# Autodesk Inventor assembly: CoreXY_Unit_Asem
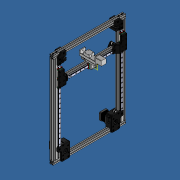
[picture p0: Inventor's stored thumbnail of the model, 180x180]
Saved by Autodesk Inventor 2020 (Build 240168000, 168)
## iProperties
Created: 2020-09-22
Part Number: CoreXY_Unit_Asem
Document SubType Name: Assembly
Designer: magnarecta
Author: magnarecta
## Documents named in this file (28)
- D:\Document\Github\CoreXY_Laser\Model\Asem\CoreXY_Unit_Asem.iam
- D:\Document\Github\CoreXY_Laser\Model\Parts\Linear_Guide\MGN12H_400mm\MGN12H_400mm.iam
- D:\Document\Github\CoreXY_Laser\Model\Parts\MISUMI\HFS5-2020-300_Autodesk_Inventor_2020_20200923\HFS5-2020-300.ipt
- D:\Document\Github\CoreXY_Laser\Model\Parts\MISUMI\HFS5-2020-420-Z5-XA10-XB30-XC390-XD410_Autodesk_Inventor_2020_20200923\HFS5-2020-420-Z5-XA10-XB30-XC390-XD410.ipt
- D:\Document\Github\CoreXY_Laser\Model\Parts\Stepper Motor\NEMA17\17HS4401\17HS4401S.ipt
- D:\Document\Github\CoreXY_Laser\Model\Parts\Idler\GT2\GT2 Pulley 20T 5mm bore without\GT2 idler pulley (5 mm bore) .ipt
- D:\Document\Github\CoreXY_Laser\Model\Parts\Pulley\GT2\GT2_20t\GT2_20teeth_5bore.ipt
- D:\Document\Github\CoreXY_Laser\Model\Parts\Print_Parts\Print_Parts_C.ipt
- D:\Document\Github\CoreXY_Laser\Model\Parts\Print_Parts\Print_Parts_D.ipt
- D:\Document\Github\CoreXY_Laser\Model\Parts\Print_Parts\Print_Parts_E.ipt
- D:\Document\Github\CoreXY_Laser\Model\Parts\Print_Parts\Print_Parts_F.ipt
- D:\Document\Github\CoreXY_Laser\Model\Parts\Print_Parts\Print_Parts_I.ipt
- D:\Document\Github\CoreXY_Laser\Model\Parts\Print_Parts\Print_Parts_J.ipt
- D:\Document\Github\CoreXY_Laser\Model\Parts\MISUMI\HFS5-2020-420-AV63.5-BV356.5-Z5-XA10-XB30-XC390-XD410_Autodesk_Inventor_2020_20201005\HFS5-2020-420-AV63_5-BV356_5-Z5-XA10-XB30-XC390-XD410.ipt
- D:\Document\Github\CoreXY_Laser\Model\Parts\Bolt\M5 x 20.ipt
- D:\Document\Github\CoreXY_Laser\Model\Parts\Bolt\M3 x 8.ipt
- D:\Document\Github\CoreXY_Laser\Model\Parts\Bolt\M4 x 8.ipt
- D:\Document\Github\CoreXY_Laser\Model\Parts\Bolt\M3 x 25.ipt
- D:\Document\Github\CoreXY_Laser\Model\Parts\Bolt\M3 x 30.ipt
- D:\Document\Github\CoreXY_Laser\Model\Parts\Bolt\M4 x 10.ipt
- D:\Document\Github\CoreXY_Laser\Model\Parts\Bolt\M3 x 35.ipt
- D:\Document\Github\CoreXY_Laser\Model\Parts\Bolt\M3 x 40.ipt
- D:\Document\Github\CoreXY_Laser\Model\Parts\MISUMI\HFS5-2040-510_Autodesk_Inventor_2020_20210519\HFS5-2040-510.ipt
- D:\Document\Github\CoreXY_Laser\Model\Parts\Print_Parts\Rev3_Parts\CoreXY_A.ipt
- D:\Document\Github\CoreXY_Laser\Model\Parts\Print_Parts\Rev3_Parts\CoreXY_B.ipt
- D:\Document\Github\CoreXY_Laser\Model\Parts\Linear_Guide\MGN12H_250mm\MGN12H_250mm.iam
- D:\Document\Github\CoreXY_Laser\Model\Parts\Linear_Guide\Linear_Unit\Linear_Unit.iam
- D:\Document\Github\CoreXY_Laser\Model\Parts\Print_Parts\Rev3_Parts\Linear_Unit_Mount.ipt
## Components (87 placed, 27 different names)
1. HFS5-2040-510:1 — 角度:5
2. MGN12H_400mm:2 [sub-assembly] — Mate:4, Flush:7, Insert:122, メイト:163, 挿入:178, メイト:170, メイト:171
3. HFS5-2040-510:2
4. MGN12H_400mm:3 [sub-assembly] — Mate:30, Flush:7, Insert:119, Insert:120, 挿入:179, メイト:172
5. HFS5-2020-420-Z5-XA10-XB30-XC390-XD410:1 — Insert:30, Insert:31, Insert:32, Insert:33, メイト:158, メイト:161
6. GT2 idler pulley (5 mm bore) :11 — Mate:70, フラッシュ:36
7. Print_Parts_J:1 — Flush:32, メイト:118, メイト:119, フラッシュ:49, Insert:82, Insert:83, Insert:84, Insert:88, Insert:89, Insert:90, Insert:134
8. Print_Parts_J:2 — Flush:32, メイト:116, メイト:117, フラッシュ:48, フラッシュ:49, Insert:85, Insert:86, Insert:87, Insert:91, Insert:92, Insert:93, Insert:135
9. Print_Parts_I:3 — Mate:70, Flush:31, メイト:118, メイト:119, Insert:132
10. Print_Parts_I:4 — Mate:72, Flush:31, メイト:116, メイト:117, Insert:133
11. GT2 idler pulley (5 mm bore) :12 — Mate:72, フラッシュ:35
12. HFS5-2020-420-AV63_5-BV356_5-Z5-XA10-XB30-XC390-XD410:1 — Insert:34, Insert:35, Insert:36, Insert:37, フラッシュ:48
13. GT2 idler pulley (5 mm bore) :13 — フラッシュ:35, メイト:166, 挿入:174
14. HFS5-2020-300:1 — フラッシュ:34, メイト:165, メイト:167, メイト:168, メイト:169, 角度:4, メイト:177, フラッシュ:58
15. GT2 idler pulley (5 mm bore) :14 — 挿入:177
16. GT2 idler pulley (5 mm bore) :15 — フラッシュ:36, 挿入:176
17. GT2 idler pulley (5 mm bore) :16 — 挿入:175
18. AS 1420 - Metric M5 x 20:1 — Insert:30
19. AS 1420 - Metric M5 x 20:2 — Insert:31
20. AS 1420 - Metric M5 x 20:3 — Insert:32
21. AS 1420 - Metric M5 x 20:4 — Insert:33
22. AS 1420 - Metric M5 x 20:5 — Insert:35
23. AS 1420 - Metric M5 x 20:6 — Insert:34
24. AS 1420 - Metric M5 x 20:7 — Insert:36
25. AS 1420 - Metric M5 x 20:8 — Insert:37
26. AS 1420 - Metric M4 x 10:7 — Insert:90
27. AS 1420 - Metric M4 x 10:8 — Insert:84
28. AS 1420 - Metric M4 x 10:9 — Insert:82
29. AS 1420 - Metric M4 x 10:10 — Insert:83
30. AS 1420 - Metric M4 x 10:11 — Insert:89
31. AS 1420 - Metric M4 x 10:12 — Insert:88
32. AS 1420 - Metric M4 x 10:13 — Insert:86
33. AS 1420 - Metric M4 x 10:14 — Insert:87
34. AS 1420 - Metric M4 x 10:15 — Insert:85
35. AS 1420 - Metric M4 x 10:16 — Insert:93
36. AS 1420 - Metric M4 x 10:17 — Insert:92
37. AS 1420 - Metric M4 x 10:18 — Insert:91
38. AS 1420 - Metric M3 x 8:15 — Insert:120
39. AS 1420 - Metric M3 x 8:17 — Insert:122
40. AS 1420 - Metric M3 x 40:1 — Insert:132
41. AS 1420 - Metric M3 x 40:2 — Insert:133
42. AS 1420 - Metric M3 x 25:18 — Insert:134
43. AS 1420 - Metric M3 x 25:19 — Insert:135
44. 17HS4401S:3 — メイト:150, 挿入:168, メイト:164
45. GT2_20teeth_5bore:3
46. GT2 idler pulley (5 mm bore) :17 — 挿入:152
47. GT2 idler pulley (5 mm bore) :18
48. Print_Parts_C:2 — 挿入:152, メイト:150, メイト:158, 挿入:168, メイト:164
49. GT2 idler pulley (5 mm bore) :19 — 挿入:167
50. Print_Parts_D:2 — 挿入:167
51. AS 1420 - Metric M3 x 30:3
52. AS 1420 - Metric M4 x 8:16
53. AS 1420 - Metric M4 x 8:17
54. AS 1420 - Metric M4 x 8:18
55. AS 1420 - Metric M4 x 8:19
56. AS 1420 - Metric M4 x 8:20
57. AS 1420 - Metric M4 x 8:21
58. AS 1420 - Metric M3 x 35:5
59. AS 1420 - Metric M3 x 35:6
60. AS 1420 - Metric M3 x 25:20
61. 17HS4401S:4 — メイト:156, 挿入:169
62. GT2 idler pulley (5 mm bore) :20
63. GT2_20teeth_5bore:4
64. Print_Parts_E:2 — メイト:161, 挿入:169
65. GT2 idler pulley (5 mm bore) :21
66. GT2 idler pulley (5 mm bore) :22
67. Print_Parts_F:2 — メイト:156, メイト:163
68. AS 1420 - Metric M4 x 8:22
69. AS 1420 - Metric M4 x 8:23
70. AS 1420 - Metric M4 x 8:24
71. AS 1420 - Metric M3 x 30:4
72. AS 1420 - Metric M4 x 10:19
73. AS 1420 - Metric M4 x 10:20
74. AS 1420 - Metric M4 x 10:21
75. AS 1420 - Metric M3 x 35:7
76. AS 1420 - Metric M3 x 35:8
77. AS 1420 - Metric M3 x 25:21
78. CoreXY_A:1 — メイト:165, メイト:166, 挿入:174, 挿入:175, メイト:167, メイト:168, 挿入:178, メイト:170, メイト:171
79. CoreXY_B:1 — メイト:169, 挿入:176, 挿入:177, 挿入:179, メイト:172, メイト:178
80. Linear_Unit:1 [sub-assembly] — 角度:4, 角度:5, 挿入:182, メイト:175
81. Linear_Unit_Mount:2 — 挿入:182, メイト:175, 挿入:183, メイト:179
82. MGN12H_250mm:2 [sub-assembly] — メイト:177, フラッシュ:58, メイト:178, 挿入:183, メイト:179
83. AS 1420 - Metric M3 x 8:10 — Insert:119
84. AS 1420 - Metric M3 x 8:11
85. AS 1420 - Metric M3 x 8:12
86. AS 1420 - Metric M3 x 8:13
87. AS 1420 - Metric M3 x 8:14
## Component patterns: (5 elements, first: AS 1420 - Metric M3 x 8:10)
## Relationships (135: Insert 63, Mate 51, Flush 17, Angle 4)
- [Mate]: HFS5-2040-510:1 ↔ MGN12H_400mm:2
- [Mate]: HFS5-2040-510:1 ↔ MGN12H_400mm:2
- [Angle] (0 deg): HFS5-2040-510:1 ↔ MGN12H_400mm:2
- [Flush] (-10 mm): HFS5-2040-510:1
- Mate:4: MGN12H_400mm:2
- [Mate]: HFS5-2040-510:2 ↔ MGN12H_400mm:3
- [Mate]: HFS5-2040-510:2 ↔ MGN12H_400mm:3
- [Angle] (0 deg): HFS5-2040-510:2 ↔ MGN12H_400mm:3
- [Flush]: HFS5-2040-510:1 ↔ HFS5-2040-510:2
- [Mate]: HFS5-2040-510:1 ↔ HFS5-2020-420-Z5-XA10-XB30-XC390-XD410:1
- [Mate]: HFS5-2040-510:1 ↔ HFS5-2020-420-Z5-XA10-XB30-XC390-XD410:1
- [Mate]: HFS5-2040-510:2 ↔ HFS5-2020-420-Z5-XA10-XB30-XC390-XD410:1
- [Mate]: HFS5-2040-510:1 ↔ HFS5-2020-420-Z5-XA10-XB30-XC390-XD410:1
- [Mate]: HFS5-2040-510:2 ↔ HFS5-2020-420-Z5-XA10-XB30-XC390-XD410:1
- [Flush] (-10 mm): HFS5-2040-510:2
- Mate:30: MGN12H_400mm:3
- Flush:7: MGN12H_400mm:2 ↔ MGN12H_400mm:3
- [Mate]: HFS5-2040-510:2 ↔ Print_Parts_J:1
- [Mate]: HFS5-2040-510:1 ↔ Print_Parts_J:2
- Mate:70: GT2 idler pulley (5 mm bore) :11 ↔ Print_Parts_I:3
- Mate:72: Print_Parts_I:4 ↔ GT2 idler pulley (5 mm bore) :12
- Flush:31: Print_Parts_I:3 ↔ Print_Parts_I:4
- Flush:32: Print_Parts_J:1 ↔ Print_Parts_J:2
- [Flush]: HFS5-2040-510:2 ↔ Print_Parts_J:1
- [Mate]: HFS5-2040-510:2 ↔ HFS5-2020-420-AV63_5-BV356_5-Z5-XA10-XB30-XC390-XD410:1
- [Mate]: HFS5-2040-510:1 ↔ HFS5-2020-420-AV63_5-BV356_5-Z5-XA10-XB30-XC390-XD410:1
- [Mate]: HFS5-2040-510:1 ↔ HFS5-2020-420-AV63_5-BV356_5-Z5-XA10-XB30-XC390-XD410:1
- フラッシュ:34 [Flush] (-10 mm): HFS5-2020-300:1
- フラッシュ:35 [Flush]: GT2 idler pulley (5 mm bore) :12 ↔ GT2 idler pulley (5 mm bore) :13
- フラッシュ:36 [Flush]: GT2 idler pulley (5 mm bore) :11 ↔ GT2 idler pulley (5 mm bore) :15
- Insert:30: HFS5-2020-420-Z5-XA10-XB30-XC390-XD410:1 ↔ AS 1420 - Metric M5 x 20:1
- Insert:31: HFS5-2020-420-Z5-XA10-XB30-XC390-XD410:1 ↔ AS 1420 - Metric M5 x 20:2
- Insert:32: HFS5-2020-420-Z5-XA10-XB30-XC390-XD410:1 ↔ AS 1420 - Metric M5 x 20:3
- Insert:33: HFS5-2020-420-Z5-XA10-XB30-XC390-XD410:1 ↔ AS 1420 - Metric M5 x 20:4
- Insert:34: HFS5-2020-420-AV63_5-BV356_5-Z5-XA10-XB30-XC390-XD410:1 ↔ AS 1420 - Metric M5 x 20:6
- Insert:35: HFS5-2020-420-AV63_5-BV356_5-Z5-XA10-XB30-XC390-XD410:1 ↔ AS 1420 - Metric M5 x 20:5
- Insert:36: HFS5-2020-420-AV63_5-BV356_5-Z5-XA10-XB30-XC390-XD410:1 ↔ AS 1420 - Metric M5 x 20:7
- Insert:37: HFS5-2020-420-AV63_5-BV356_5-Z5-XA10-XB30-XC390-XD410:1 ↔ AS 1420 - Metric M5 x 20:8
- メイト:116 [Mate]: Print_Parts_J:2 ↔ Print_Parts_I:4
- メイト:117 [Mate]: Print_Parts_J:2 ↔ Print_Parts_I:4
- メイト:118 [Mate]: Print_Parts_J:1 ↔ Print_Parts_I:3
- メイト:119 [Mate]: Print_Parts_J:1 ↔ Print_Parts_I:3
- フラッシュ:48 [Flush] (-8 mm): Print_Parts_J:2 ↔ HFS5-2020-420-AV63_5-BV356_5-Z5-XA10-XB30-XC390-XD410:1
- フラッシュ:49 [Flush]: Print_Parts_J:1 ↔ Print_Parts_J:2
- Insert:82: Print_Parts_J:1 ↔ AS 1420 - Metric M4 x 10:9
- Insert:83: Print_Parts_J:1 ↔ AS 1420 - Metric M4 x 10:10
- Insert:84: Print_Parts_J:1 ↔ AS 1420 - Metric M4 x 10:8
- Insert:85: Print_Parts_J:2 ↔ AS 1420 - Metric M4 x 10:15
- Insert:86: Print_Parts_J:2 ↔ AS 1420 - Metric M4 x 10:13
- Insert:87: Print_Parts_J:2 ↔ AS 1420 - Metric M4 x 10:14
- Insert:88: Print_Parts_J:1 ↔ AS 1420 - Metric M4 x 10:12
- Insert:89: Print_Parts_J:1 ↔ AS 1420 - Metric M4 x 10:11
- Insert:90: Print_Parts_J:1 ↔ AS 1420 - Metric M4 x 10:7
- Insert:91: Print_Parts_J:2 ↔ AS 1420 - Metric M4 x 10:18
- Insert:92: Print_Parts_J:2 ↔ AS 1420 - Metric M4 x 10:17
- Insert:93: Print_Parts_J:2 ↔ AS 1420 - Metric M4 x 10:16
- Insert:119: MGN12H_400mm:3 ↔ AS 1420 - Metric M3 x 8:10
- Insert:120: MGN12H_400mm:3 ↔ AS 1420 - Metric M3 x 8:15
- Insert:122: MGN12H_400mm:2 ↔ AS 1420 - Metric M3 x 8:17
- Insert:132: Print_Parts_I:3 ↔ AS 1420 - Metric M3 x 40:1
- Insert:133: Print_Parts_I:4 ↔ AS 1420 - Metric M3 x 40:2
- Insert:134: Print_Parts_J:1 ↔ AS 1420 - Metric M3 x 25:18
- Insert:135: Print_Parts_J:2 ↔ AS 1420 - Metric M3 x 25:19
- [Mate]: 17HS4401S:3 ↔ GT2_20teeth_5bore:3
- [Flush]: GT2 idler pulley (5 mm bore) :17 ↔ GT2 idler pulley (5 mm bore) :18
- [Mate]: GT2 idler pulley (5 mm bore) :17 ↔ GT2 idler pulley (5 mm bore) :19
- [Insert]: Print_Parts_C:2 ↔ Print_Parts_D:2
- [Mate]: Print_Parts_C:2 ↔ Print_Parts_D:2
- [Flush]: GT2_20teeth_5bore:3 ↔ GT2 idler pulley (5 mm bore) :18
- [Insert]: Print_Parts_D:2 ↔ AS 1420 - Metric M3 x 30:3
- [Insert]: Print_Parts_C:2 ↔ AS 1420 - Metric M4 x 8:16
- [Insert]: Print_Parts_C:2 ↔ AS 1420 - Metric M4 x 8:17
- [Insert]: Print_Parts_C:2 ↔ AS 1420 - Metric M4 x 8:18
- [Insert]: Print_Parts_D:2 ↔ AS 1420 - Metric M4 x 8:21
- [Insert]: Print_Parts_D:2 ↔ AS 1420 - Metric M4 x 8:20
- [Insert]: Print_Parts_D:2 ↔ AS 1420 - Metric M4 x 8:19
- [Insert]: Print_Parts_D:2 ↔ AS 1420 - Metric M3 x 35:5
- [Insert]: Print_Parts_D:2 ↔ AS 1420 - Metric M3 x 35:6
- [Insert]: Print_Parts_D:2 ↔ AS 1420 - Metric M3 x 25:20
- 挿入:152 [Insert]: GT2 idler pulley (5 mm bore) :17 ↔ Print_Parts_C:2
- メイト:150 [Mate]: 17HS4401S:3 ↔ Print_Parts_C:2
- [Mate]: 17HS4401S:4 ↔ GT2_20teeth_5bore:4
- [Mate]: GT2 idler pulley (5 mm bore) :21 ↔ GT2 idler pulley (5 mm bore) :22
- [Flush]: GT2 idler pulley (5 mm bore) :20 ↔ GT2 idler pulley (5 mm bore) :22
- [Mate]: Print_Parts_E:2 ↔ Print_Parts_F:2
- [Mate]: Print_Parts_E:2 ↔ Print_Parts_F:2
- [Insert]: Print_Parts_E:2 ↔ Print_Parts_F:2
- [Insert]: GT2 idler pulley (5 mm bore) :22 ↔ Print_Parts_F:2
- [Insert]: Print_Parts_E:2 ↔ GT2 idler pulley (5 mm bore) :21
- [Flush]: GT2_20teeth_5bore:4 ↔ GT2 idler pulley (5 mm bore) :22
- [Insert]: Print_Parts_E:2 ↔ AS 1420 - Metric M4 x 8:22
- [Insert]: Print_Parts_E:2 ↔ AS 1420 - Metric M4 x 8:23
- [Insert]: Print_Parts_E:2 ↔ AS 1420 - Metric M4 x 8:24
- [Insert]: Print_Parts_F:2 ↔ AS 1420 - Metric M3 x 30:4
- [Insert]: Print_Parts_F:2 ↔ AS 1420 - Metric M4 x 10:21
- [Insert]: Print_Parts_F:2 ↔ AS 1420 - Metric M4 x 10:19
- [Insert]: Print_Parts_F:2 ↔ AS 1420 - Metric M4 x 10:20
- [Insert]: Print_Parts_F:2 ↔ AS 1420 - Metric M3 x 35:7
- [Insert]: Print_Parts_F:2 ↔ AS 1420 - Metric M3 x 35:8
- [Insert]: Print_Parts_F:2 ↔ AS 1420 - Metric M3 x 25:21
- メイト:156 [Mate]: 17HS4401S:4 ↔ Print_Parts_F:2
- 挿入:167 [Insert]: GT2 idler pulley (5 mm bore) :19 ↔ Print_Parts_D:2
- [Mate]: HFS5-2040-510:2 ↔ Print_Parts_C:2
- メイト:158 [Mate]: HFS5-2020-420-Z5-XA10-XB30-XC390-XD410:1 ↔ Print_Parts_C:2
- [Mate]: HFS5-2040-510:2 ↔ Print_Parts_C:2
- [Mate]: HFS5-2040-510:1 ↔ Print_Parts_E:2
- メイト:161 [Mate]: HFS5-2020-420-Z5-XA10-XB30-XC390-XD410:1 ↔ Print_Parts_E:2
- [Mate]: HFS5-2040-510:1 ↔ Print_Parts_E:2
- メイト:163 [Mate]: MGN12H_400mm:2 ↔ Print_Parts_F:2
- 挿入:168 [Insert]: 17HS4401S:3 ↔ Print_Parts_C:2
- メイト:164 [Mate]: 17HS4401S:3 ↔ Print_Parts_C:2
- 挿入:169 [Insert]: 17HS4401S:4 ↔ Print_Parts_E:2
- メイト:165 [Mate]: HFS5-2020-300:1 ↔ CoreXY_A:1
- メイト:166 [Mate]: GT2 idler pulley (5 mm bore) :13 ↔ CoreXY_A:1
- 挿入:174 [Insert] (0.1 mm): GT2 idler pulley (5 mm bore) :13 ↔ CoreXY_A:1
- 挿入:175 [Insert] (0.1 mm): GT2 idler pulley (5 mm bore) :16 ↔ CoreXY_A:1
- メイト:167 [Mate]: HFS5-2020-300:1 ↔ CoreXY_A:1
- メイト:168 [Mate] (0.1 mm): HFS5-2020-300:1 ↔ CoreXY_A:1
- メイト:169 [Mate]: HFS5-2020-300:1 ↔ CoreXY_B:1
- 挿入:176 [Insert] (0.1 mm): GT2 idler pulley (5 mm bore) :15 ↔ CoreXY_B:1
- 挿入:177 [Insert] (0.1 mm): GT2 idler pulley (5 mm bore) :14 ↔ CoreXY_B:1
- 挿入:178 [Insert]: MGN12H_400mm:2 ↔ CoreXY_A:1
- メイト:170 [Mate]: MGN12H_400mm:2 ↔ CoreXY_A:1
- メイト:171 [Mate]: MGN12H_400mm:2 ↔ CoreXY_A:1
- 挿入:179 [Insert]: MGN12H_400mm:3 ↔ CoreXY_B:1
- メイト:172 [Mate]: MGN12H_400mm:3 ↔ CoreXY_B:1
- 角度:4 [Angle] (180 deg): HFS5-2020-300:1 ↔ Linear_Unit:1
- 角度:5 [Angle] (0 deg): HFS5-2040-510:1 ↔ Linear_Unit:1
- 挿入:182 [Insert]: Linear_Unit:1 ↔ Linear_Unit_Mount:2
- メイト:175 [Mate]: Linear_Unit:1 ↔ Linear_Unit_Mount:2
- メイト:177 [Mate]: HFS5-2020-300:1 ↔ MGN12H_250mm:2
- フラッシュ:58 [Flush] (-4 mm): HFS5-2020-300:1 ↔ MGN12H_250mm:2
- メイト:178 [Mate] (5 mm): CoreXY_B:1 ↔ MGN12H_250mm:2
- 挿入:183 [Insert]: Linear_Unit_Mount:2 ↔ MGN12H_250mm:2
- メイト:179 [Mate]: Linear_Unit_Mount:2 ↔ MGN12H_250mm:2
## Named parameters: d36_d6 = 0 deg, d37_d3 = 0 mm, d38_d5 = 0 mm, d548_d356 = 0 mm, d549_d357 = 0 mm, d550_d359 = 0 mm, d551_d341 = 0 mm, d552_d342 = 0 mm, d553_d343 = 0 mm, d554_d344 = 0 mm, d555_d345 = 0 mm, d556_d346 = 0 mm, d557_d321 = 0 mm, d558_d210 = 0 mm, d559_d100 = 0 mm, d560_d102 = 0 mm, d561_d103 = 0 mm, d562_d79 = 0 mm, d563_d87 = 0 mm, d569_d355 = 0 mm, d570_d358 = 0 mm, d571_d327 = 0 mm, d572_d328 = 0 mm, d573_d329 = 0 mm, d574_d354 = 0 mm, d575_d309 = 0 mm, d576_d310 = 0 mm, d577_d311 = 0 mm, d578_d320 = 0 mm, d579_d211 = 0 mm, d580_d202 = 0 mm, d581_d203 = 0 mm, d583_d107_d100 = 0 mm, d585_d112 = 0 mm, d586_d113 = 0 mm, d587_d114 = 0 mm, d588_d115 = 0 mm, d589_d81 = 0 mm
